# Autodesk Inventor assembly: Random Thing
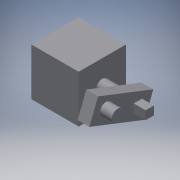
[picture p0: Inventor's stored thumbnail of the model, 180x180]
Saved by Autodesk Inventor 2019 (Build 230136000, 136)
## iProperties
Created: 2019-04-11
Part Number: Random Thing
Document SubType Name: Assembly
Designer: User
Author: User
## Documents named in this file (5)
- C:\Robotics\CAD\2019-20_CAD\offseason\random ideas\Random Thing.iam
- C:\Robotics\CAD\2019-20_CAD\offseason\random ideas\Cube.ipt
- C:\Robotics\CAD\2019-20_CAD\offseason\random ideas\Peg.ipt
- C:\Robotics\CAD\2019-20_CAD\offseason\random ideas\Switch.ipt
- C:\Robotics\CAD\2019-20_CAD\offseason\random ideas\Another_Button.ipt
## Components (4 placed, 4 different names)
1. Cube:1
2. Peg:1 — Insert:1
3. Switch:1 — Insert:1, Mate:1
4. Another_Button:1 — Mate:1
## Relationships (2: Insert 1, Mate 1)
- Insert:1: Peg:1 ↔ Switch:1
- Mate:1: Switch:1 ↔ Another_Button:1
